# Autodesk Inventor assembly: roller cage_MIR
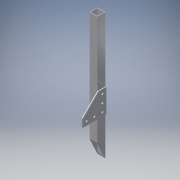
[picture p0: Inventor's stored thumbnail of the model, 180x180]
Saved by Autodesk Inventor 2016 (Build 200138000, 138)
## iProperties
Created: 2016-02-02
Part Number: roller cage_MIR
Document SubType Name: Assembly
Designer: gus
Mass: 119.442 g
Surface Area: 1363.6 cm^2
Volume: 119.442 cm^3
Density: 1 g/cm^3
Author: gus
## Documents named in this file (5)
- \\Mac\Home\Desktop\1510-stronghold-CAD-master\roller cage\roller cage_MIR.iam
- \\Mac\Home\Desktop\1510-stronghold-CAD-master\roller cage\top_MIR.ipt
- \\Mac\Home\Desktop\1510-stronghold-CAD-master\roller cage\gusset plate_MIR.ipt
- \\Mac\Home\Desktop\1510-stronghold-CAD-master\roller cage\robot_MIR.iam
- \\Mac\Home\Desktop\1510-stronghold-CAD-master\roller cage\ramp gusset_MIR.ipt
## Components (5 placed, 4 different names)
1. top_MIR:1 — Mate:8, Mate:7, Mate:3, Mate:6, Mate:5, Mate:4, Mate:11, Mate:10, Mate:9
2. gusset plate_MIR:1 — Mate:8, Mate:7, Mate:3
3. robot_MIR:1 [sub-assembly]
4. ramp gusset_MIR:1 — Mate:6, Mate:5, Mate:4
5. gusset plate_MIR:2 — Mate:11, Mate:10, Mate:9
## Relationships (9: Mate 9)
- Mate:8: top_MIR:1 ↔ gusset plate_MIR:1
- Mate:7: top_MIR:1 ↔ gusset plate_MIR:1
- Mate:3: top_MIR:1 ↔ gusset plate_MIR:1
- Mate:6: top_MIR:1 ↔ ramp gusset_MIR:1
- Mate:5: top_MIR:1 ↔ ramp gusset_MIR:1
- Mate:4: top_MIR:1 ↔ ramp gusset_MIR:1
- Mate:11: top_MIR:1 ↔ gusset plate_MIR:2
- Mate:10: top_MIR:1 ↔ gusset plate_MIR:2
- Mate:9: top_MIR:1 ↔ gusset plate_MIR:2
